(part 1 of 2)
# Autodesk Inventor assembly: ELEV_000_FULLASMBLY
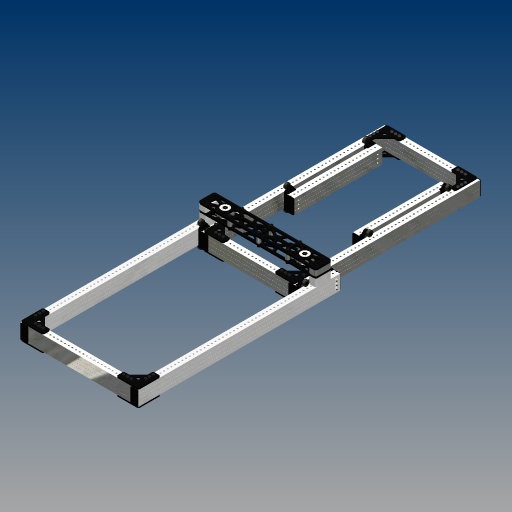
[picture p0: Inventor's stored thumbnail of the model, 512x512]
Saved by Autodesk Inventor 2024.3 (Build 283343000, 343)
## iProperties
Created: 2024-11-25
Part Number: ELEV_000_FULLASMBLY
Document SubType Name: Assembly
Designer: Kenji
Mass: 3407.89 g
Surface Area: 12378 cm^2
Volume: 1206.36 cm^3
Density: 2.82493 g/cm^3
Author: Kenji
## Documents named in this file (36)
- C:\Users\Kenji\Documents\GitHub\1622-2024-Casino-Clash-CAD-A-Thon\Elevator\ELEV_000_FULLASMBLY.iam
- C:\Users\Kenji\Documents\GitHub\1622-2024-Casino-Clash-CAD-A-Thon\Elevator\ELEV_001_BAR1(27.500 in).ipt
- C:\Users\Kenji\Documents\GitHub\1622-2024-Casino-Clash-CAD-A-Thon\Elevator\ELEV_002_BAR2(14.000 in).ipt
- C:\Users\Kenji\Documents\GitHub\1622-2024-Casino-Clash-CAD-A-Thon\Elevator\ELEV_003_BAR3(25.000 in).ipt
- C:\Users\Kenji\Documents\GitHub\1622-2024-Casino-Clash-CAD-A-Thon\COTS Library\Motion\BearingBlocks\ElevatorBlocks\WCP-0897_InlineBearingBlock.iam
- C:\Users\Kenji\Documents\GitHub\1622-2024-Casino-Clash-CAD-A-Thon\Elevator\ELEV_004_BAR4(12.000 in).ipt
- C:\Users\Kenji\Documents\GitHub\1622-2024-Casino-Clash-CAD-A-Thon\Elevator\ELEV_005_SUPBRK1.ipt
- C:\Users\Kenji\Documents\GitHub\1622-2024-Casino-Clash-CAD-A-Thon\COTS Library\Fasteners\Nuts\COTS_90633A411_Low-Strength Steel Thin Nylon-Insert Locknut_10-32.ipt
- C:\Users\Kenji\Documents\GitHub\1622-2024-Casino-Clash-CAD-A-Thon\Elevator\ELEV_006_SUPBRK1_THRD.ipt
- C:\Users\Kenji\Documents\GitHub\1622-2024-Casino-Clash-CAD-A-Thon\COTS Library\Fasteners\Bolts\Socket-Head\10-32\COTS_90044A121_Black-Oxide Alloy Steel Socket Head Screw_10-32_2.5in.ipt
- C:\Users\Kenji\Documents\GitHub\1622-2024-Casino-Clash-CAD-A-Thon\COTS Library\Fasteners\Bolts\Socket-Head\10-32\COTS_90044A202_Black-Oxide Alloy Steel Socket Head Screw_1-.375.ipt
- C:\Users\Kenji\Documents\GitHub\1622-2024-Casino-Clash-CAD-A-Thon\COTS Library\Fasteners\Bolts\Socket-Head\10-32\COTS_91251A342_Black-Oxide Alloy Steel Socket Head Screw_.5in.ipt
- C:\Users\Kenji\Documents\GitHub\1622-2024-Casino-Clash-CAD-A-Thon\Elevator\ELEV_007_SUPBRK2.ipt
- C:\Users\Kenji\Documents\GitHub\1622-2024-Casino-Clash-CAD-A-Thon\COTS Library\Fasteners\Bolts\Socket-Head\10-32\COTS_91251A359_Black-Oxide Alloy Steel Socket Head Screw_10-32_2_3-4in.ipt
- C:\Users\Kenji\Documents\GitHub\1622-2024-Casino-Clash-CAD-A-Thon\COTS Library\Fasteners\Nuts\COTS_90631A411_Low-Strength Steel Nylon-Insert Locknut_10-32.ipt
- C:\Users\Kenji\Documents\GitHub\1622-2024-Casino-Clash-CAD-A-Thon\Elevator\ELEV_008_SUPBRK3.ipt
- C:\Users\Kenji\Documents\GitHub\1622-2024-Casino-Clash-CAD-A-Thon\Elevator\ELEV_010_BOLTCOVER2.ipt
- C:\Users\Kenji\Documents\GitHub\1622-2024-Casino-Clash-CAD-A-Thon\Elevator\ELEV_011_EXTRUENDCAP.ipt
- C:\Users\Kenji\Documents\GitHub\1622-2024-Casino-Clash-CAD-A-Thon\Elevator\ELEV_012_SUPBRK2_THRD.ipt
- C:\Users\Kenji\Documents\GitHub\1622-2024-Casino-Clash-CAD-A-Thon\Elevator\ELEV_013_BAR5(12.000 in).ipt
- C:\Users\Kenji\Documents\GitHub\1622-2024-Casino-Clash-CAD-A-Thon\Elevator\ELEV_015_CRSHBLCK1.ipt
- C:\Users\Kenji\Documents\GitHub\1622-2024-Casino-Clash-CAD-A-Thon\Elevator\ELEV_019_SUPBAR3.ipt
- C:\Users\Kenji\Documents\GitHub\1622-2024-Casino-Clash-CAD-A-Thon\COTS Library\Motion\Bearings\COTS_WCP-0783_1.125ODHexBearing.ipt
- C:\Users\Kenji\Documents\GitHub\1622-2024-Casino-Clash-CAD-A-Thon\COTS Library\Motion\Sprockets\COTS_WCP-0974_#35_15t.ipt
- C:\Users\Kenji\Documents\GitHub\1622-2024-Casino-Clash-CAD-A-Thon\Elevator\ELEV_020_BILLET1(Shit).ipt
- C:\Users\Kenji\Documents\GitHub\1622-2024-Casino-Clash-CAD-A-Thon\Elevator\ELEV_021_SPACER2.ipt
- C:\Users\Kenji\Documents\GitHub\1622-2024-Casino-Clash-CAD-A-Thon\Elevator\ELEV_022_WASHER1(3DP).ipt
- C:\Users\Kenji\Documents\GitHub\1622-2024-Casino-Clash-CAD-A-Thon\COTS Library\Fasteners\Bolts\Socket-Head\0.25-20\COTS_91251A537_Black-Oxide Alloy Steel Socket Head Screw_.25-20_.5in.ipt
- C:\Users\Kenji\Documents\GitHub\1622-2024-Casino-Clash-CAD-A-Thon\Elevator\ELEV_023_BILLET2.ipt
- C:\Users\Kenji\Documents\GitHub\1622-2024-Casino-Clash-CAD-A-Thon\Elevator\ELEV_024_SPACER1.ipt
- C:\Users\Kenji\Documents\GitHub\1622-2024-Casino-Clash-CAD-A-Thon\Elevator\ELEV_000_FULLASMBLY\AIP\FEA\ew6g7bhkw.fins
- C:\Users\Kenji\Documents\GitHub\1622-2024-Casino-Clash-CAD-A-Thon\Elevator\ELEV_000_FULLASMBLY\AIP\FEA\ew6g7bhkw.fsat
- C:\Users\Kenji\Documents\GitHub\1622-2024-Casino-Clash-CAD-A-Thon\Elevator\ELEV_000_FULLASMBLY\AIP\FEA\ew6g7bhkw.ftes
- C:\Users\Kenji\Documents\GitHub\1622-2024-Casino-Clash-CAD-A-Thon\Elevator\ELEV_000_FULLASMBLY\AIP\FEA\ew6g7bhkw.fwiz
- C:\Users\Kenji\Documents\GitHub\1622-2024-Casino-Clash-CAD-A-Thon\Elevator\ELEV_000_FULLASMBLY\AIP\FEA\ew6g7biao.fmsh
- C:\Users\Kenji\Documents\GitHub\1622-2024-Casino-Clash-CAD-A-Thon\Elevator\ELEV_000_FULLASMBLY\AIP\FEA\ew6g7bibk.fres
## Components (210 placed, 29 different names)
1. ELEV_001_BAR1(27.500 in):1 — Flush:1, Flush:2, Mate:1, Mate:2, Flush:7, Tangent:2, Mate:10, Flush:11, Mate:11, Mate:78, Mate:133, Mate:136, Mate:137, Mate:201, Mate:202, Mate:203, Mate:284, Mate:285, Mate:286, Flush:35, Mate:341, Mate:359
2. ELEV_001_BAR1(27.500 in):2 — Flush:1, Flush:2, Mate:1, Flush:3, Flush:4, Mate:3, Angle:1, Mate:4, Flush:8, Angle:2, Mate:74, Mate:128, Mate:131, Mate:198, Mate:199, Mate:200, Mate:287, Mate:288, Mate:289, Mate:363
3. ELEV_002_BAR2(14.000 in):1 — Flush:3, Flush:4, Mate:2, Mate:127, Flush:24, Mate:132, Mate:134, Mate:135
4. ELEV_003_BAR3(25.000 in):1 — Flush:5, Flush:6, Flush:7, Mate:8, Flush:10, Mate:9, Mate:82, Mate:186, Mate:187, Mate:188, Mate:211, Mate:228, Tangent:3, Tangent:4, Angle:5, Angle:6, Mate:265, Mate:266, Mate:267
5. ELEV_003_BAR3(25.000 in):2 — Flush:5, Flush:6, Tangent:1, Angle:2, Mate:5, Angle:3, Mate:6, Flush:9, Mate:12, Flush:12, Flush:13, Mate:13, Flush:14, Mate:14, Mate:16, Mate:62, Mate:86, Mate:189, Mate:190, Mate:191, Mate:192, Mate:193, Mate:194, Mate:207, Mate:208, Tangent:5, Flush:33
6. WCP-0897_InlineBearingBlock:1 [sub-assembly] — Mate:5, Angle:3, Mate:6, Flush:9, Mate:83, Mate:84
7. WCP-0897_InlineBearingBlock:2 [sub-assembly] — Mate:3, Angle:1, Mate:4, Tangent:1, Flush:8, Mate:71, Mate:72
8. WCP-0897_InlineBearingBlock:3 [sub-assembly] — Mate:8, Flush:10, Mate:9, Tangent:2, Mate:79, Mate:80
9. WCP-0897_InlineBearingBlock:4 [sub-assembly] — Mate:10, Flush:11, Mate:11, Mate:75, Mate:76
10. ELEV_004_BAR4(12.000 in):1 — Mate:12, Flush:12, Flush:13, Mate:17, Mate:18, Mate:19, Angle:4, Mate:20, Mate:42, Mate:45, Mate:60, Flush:15, Mate:61
11. ELEV_004_BAR4(12.000 in):2 — Mate:13, Flush:14, Mate:14, Flush:26, Flush:27, Mate:214, Mate:227, Flush:28, Angle:7
12. ELEV_005_SUPBRK1:1 — Mate:16, Mate:17, Mate:18, Mate:67, Mate:68, Mate:69, Mate:70
13. ELEV_005_SUPBRK1:2 — Mate:19, Angle:4, Mate:20, Mate:63, Mate:64, Mate:65, Mate:66
14. ELEV_006_SUPBRK1_THRD:1 — Mate:42, Mate:61, Mate:62, Mate:247, Mate:248
15. ELEV_006_SUPBRK1_THRD:2 — Mate:45, Mate:60, Flush:15, Mate:241, Mate:242, Mate:243, Mate:244
16. ELEV_008_SUPBRK3:1 — Mate:127, Flush:24, Mate:128, Mate:129, Mate:130, Mate:138, Mate:139, Mate:144, Mate:145
17. ELEV_008_SUPBRK3:2 — Mate:129, Mate:130, Mate:131, Mate:148, Mate:149
18. ELEV_008_SUPBRK3:3 — Mate:132, Mate:133, Mate:134, Mate:151, Mate:153
19. ELEV_008_SUPBRK3:4 — Mate:135, Mate:136, Mate:137, Mate:140, Mate:141, Mate:142, Mate:143
20. ELEV_011_EXTRUENDCAP:1 — Mate:189, Mate:190, Mate:191
21. ELEV_011_EXTRUENDCAP:3 — Mate:186, Mate:187, Mate:188
22. ELEV_011_EXTRUENDCAP:5 — Mate:198, Mate:199, Mate:200
23. ELEV_011_EXTRUENDCAP:6 — Mate:201, Mate:202, Mate:203
24. ELEV_011_EXTRUENDCAP:7 — Mate:192, Mate:193, Mate:194
25. ELEV_007_SUPBRK2:1 — Flush:26, Mate:227, Mate:228, Mate:229, Mate:230, Mate:231, Mate:232, Mate:233
26. ELEV_007_SUPBRK2:2 — Flush:27, Mate:207, Mate:208, Mate:212, Mate:213, Mate:217, Mate:218, Mate:219, Mate:220
27. ELEV_012_SUPBRK2_THRD:1 — Mate:211, Mate:229, Flush:28, Mate:239, Mate:240
28. ELEV_012_SUPBRK2_THRD:2 — Mate:212, Mate:213, Mate:214, Mate:235, Mate:332
29. ELEV_013_BAR5(12.000 in):1 — Mate:257, Flush:29, Mate:258, Mate:259, Flush:30, Mate:260, Angle:5, Angle:6, Flush:34, Mate:277, Mate:283, Mate:333, Mate:334, Mate:335
30. ELEV_013_BAR5(12.000 in):2 — Mate:261, Flush:31, Mate:262, Mate:263, Flush:32, Mate:264, Angle:7, Flush:33, Flush:34, Mate:279, Mate:281, Mate:336, Mate:337, Mate:338
31. WCP-0897_InlineBearingBlock:5 [sub-assembly] — Mate:257, Flush:29, Mate:258, Tangent:3, Tangent:4, Mate:270, Mate:271
32. WCP-0897_InlineBearingBlock:6 [sub-assembly] — Mate:259, Flush:30, Mate:260, Mate:274, Mate:275
33. WCP-0897_InlineBearingBlock:7 [sub-assembly] — Mate:261, Flush:31, Mate:262, Tangent:5, Mate:272, Mate:273
34. WCP-0897_InlineBearingBlock:8 [sub-assembly] — Mate:263, Flush:32, Mate:264, Mate:268, Mate:269
35. ELEV_011_EXTRUENDCAP:8 — Mate:265, Mate:266, Mate:267
36. ELEV_015_CRSHBLCK1:1 — Mate:284, Mate:285, Mate:286
37. ELEV_015_CRSHBLCK1:2 — Mate:287, Mate:288, Mate:289
38. ELEV_011_EXTRUENDCAP:9 — Mate:333, Mate:334, Mate:335
39. ELEV_011_EXTRUENDCAP:10 — Mate:336, Mate:337, Mate:338
40. ELEV_019_SUPBAR3:1 — Flush:35, Mate:341, Mate:342, Mate:343, Mate:344, Mate:345, Mate:348, Mate:349, Mate:357, Mate:358, Mate:364, Mate:365, Mate:366, Mate:367, Mate:368, Mate:369, Mate:370, Mate:371, Mate:374, Mate:386, Mate:387, Mate:388, Mate:389, Mate:390, Mate:391, Mate:392, Mate:393, Mate:394, Mate:395, Mate:396, Mate:397, Mate:410, Mate:411, Mate:412, Mate:415
41. ELEV_019_SUPBAR3:2 — Mate:342, Mate:343, Mate:346, Mate:347, Mate:350, Mate:351, Mate:360, Mate:361, Mate:362, Mate:372, Mate:373, Mate:375, Mate:376, Mate:398, Mate:399, Mate:400, Mate:401, Mate:402, Mate:403, Mate:404, Mate:405, Mate:406, Mate:407, Mate:408, Mate:409, Mate:413, Mate:414
42. COTS_WCP-0783_1.125ODHexBearing:1 — Mate:347, Mate:350, Mate:352, Angle:11, Mate:383
43. COTS_WCP-0783_1.125ODHexBearing:2 — Mate:345, Mate:349, Angle:10, Mate:380, Mate:381, Mate:382, Mate:417, Angle:13, Flush:37
44. COTS_WCP-0783_1.125ODHexBearing:3 — Mate:346, Mate:351, Angle:9
45. COTS_WCP-0783_1.125ODHexBearing:4 — Mate:344, Mate:348, Mate:353, Angle:8, Mate:378, Mate:416, Angle:12, Flush:36
46. COTS_WCP-0974_#35_15t:1 — Mate:352, Angle:10, Angle:11, Mate:385
47. COTS_WCP-0974_#35_15t:2 — Mate:353, Angle:8, Angle:9, Mate:377, Mate:379, Mate:384
48. ELEV_020_BILLET1(Shit):1 — Mate:357, Mate:358, Mate:359, Mate:360
49. ELEV_020_BILLET1(Shit):2 — Mate:361, Mate:362, Mate:363
50. ELEV_021_SPACER2:1 — Mate:368, Mate:371
51. ELEV_021_SPACER2:2 — Mate:367, Mate:375
52. ELEV_021_SPACER2:3 — Mate:366, Mate:374, Mate:376
53. ELEV_021_SPACER2:4 — Mate:365, Mate:373
54. ELEV_021_SPACER2:5 — Mate:364, Mate:372
55. ELEV_021_SPACER2:6 — Mate:369, Mate:370
56. ELEV_022_WASHER1(3DP):1 — Mate:381, Mate:382, Mate:385
57. ELEV_022_WASHER1(3DP):2 — Mate:380, Mate:383
58. ELEV_022_WASHER1(3DP):3 — Mate:377, Mate:378
59. ELEV_022_WASHER1(3DP):4 — Mate:379, Mate:384
60. COTS_91251A537_Black-Oxide Alloy Steel Socket Head Screw_.25-20_.5in:1 — Mate:386, Mate:396
61. COTS_91251A537_Black-Oxide Alloy Steel Socket Head Screw_.25-20_.5in:2 — Mate:387, Mate:397
62. COTS_91251A537_Black-Oxide Alloy Steel Socket Head Screw_.25-20_.5in:3 — Mate:388, Mate:394
63. COTS_91251A537_Black-Oxide Alloy Steel Socket Head Screw_.25-20_.5in:4 — Mate:389, Mate:395
64. COTS_91251A537_Black-Oxide Alloy Steel Socket Head Screw_.25-20_.5in:5 — Mate:390, Mate:392
65. COTS_91251A537_Black-Oxide Alloy Steel Socket Head Screw_.25-20_.5in:6 — Mate:391, Mate:393
66. COTS_91251A537_Black-Oxide Alloy Steel Socket Head Screw_.25-20_.5in:7 — Mate:399, Mate:405
67. COTS_91251A537_Black-Oxide Alloy Steel Socket Head Screw_.25-20_.5in:8 — Mate:400, Mate:406
68. COTS_91251A537_Black-Oxide Alloy Steel Socket Head Screw_.25-20_.5in:9 — Mate:401, Mate:407
69. COTS_91251A537_Black-Oxide Alloy Steel Socket Head Screw_.25-20_.5in:10 — Mate:402, Mate:408
70. COTS_91251A537_Black-Oxide Alloy Steel Socket Head Screw_.25-20_.5in:11 — Mate:398, Mate:404
71. COTS_91251A537_Black-Oxide Alloy Steel Socket Head Screw_.25-20_.5in:12 — Mate:403, Mate:409
72. ELEV_023_BILLET2:1 — Mate:410, Mate:411, Mate:412
73. ELEV_023_BILLET2:2 — Mate:413, Mate:414, Mate:415
74. ELEV_024_SPACER1:1 — Mate:416, Angle:12, Flush:36
75. ELEV_024_SPACER1:2 — Mate:417, Angle:13, Flush:37
76. COTS_90044A121_Black-Oxide Alloy Steel Socket Head Screw_10-32_2.5in:1 — Mate:63, Mate:64
77. COTS_90044A121_Black-Oxide Alloy Steel Socket Head Screw_10-32_2.5in:5
78. COTS_90044A121_Black-Oxide Alloy Steel Socket Head Screw_10-32_2.5in:6
79. COTS_90044A121_Black-Oxide Alloy Steel Socket Head Screw_10-32_2.5in:4 — Mate:65, Mate:66
80. COTS_90044A121_Black-Oxide Alloy Steel Socket Head Screw_10-32_2.5in:7
81. COTS_90044A121_Black-Oxide Alloy Steel Socket Head Screw_10-32_2.5in:8
82. COTS_90044A121_Black-Oxide Alloy Steel Socket Head Screw_10-32_2.5in:2 — Mate:67, Mate:69, Mate:245
83. COTS_90044A121_Black-Oxide Alloy Steel Socket Head Screw_10-32_2.5in:11
84. COTS_90044A121_Black-Oxide Alloy Steel Socket Head Screw_10-32_2.5in:12
85. COTS_90044A202_Black-Oxide Alloy Steel Socket Head Screw_1-.375:1 — Mate:71, Mate:72, Mate:73
86. COTS_90633A411_Low-Strength Steel Thin Nylon-Insert Locknut_10-32:1 — Mate:73, Mate:74
87. COTS_90044A202_Black-Oxide Alloy Steel Socket Head Screw_1-.375:2
88. COTS_90633A411_Low-Strength Steel Thin Nylon-Insert Locknut_10-32:2
89. COTS_90044A202_Black-Oxide Alloy Steel Socket Head Screw_1-.375:3
90. COTS_90633A411_Low-Strength Steel Thin Nylon-Insert Locknut_10-32:3
91. COTS_90633A411_Low-Strength Steel Thin Nylon-Insert Locknut_10-32:4 — Mate:77, Mate:78
92. COTS_90044A202_Black-Oxide Alloy Steel Socket Head Screw_1-.375:4 — Mate:75, Mate:76, Mate:77
93. COTS_90633A411_Low-Strength Steel Thin Nylon-Insert Locknut_10-32:5
94. COTS_90044A202_Black-Oxide Alloy Steel Socket Head Screw_1-.375:5
95. COTS_90633A411_Low-Strength Steel Thin Nylon-Insert Locknut_10-32:6
96. COTS_90044A202_Black-Oxide Alloy Steel Socket Head Screw_1-.375:6
97. COTS_91251A342_Black-Oxide Alloy Steel Socket Head Screw_.5in:1 — Mate:79, Mate:80, Mate:81
98. COTS_90633A411_Low-Strength Steel Thin Nylon-Insert Locknut_10-32:7 — Mate:81, Mate:82
99. COTS_91251A342_Black-Oxide Alloy Steel Socket Head Screw_.5in:2
100. COTS_90633A411_Low-Strength Steel Thin Nylon-Insert Locknut_10-32:8
101. COTS_91251A342_Black-Oxide Alloy Steel Socket Head Screw_.5in:3
102. COTS_90633A411_Low-Strength Steel Thin Nylon-Insert Locknut_10-32:9
103. COTS_90633A411_Low-Strength Steel Thin Nylon-Insert Locknut_10-32:10 — Mate:85, Mate:86
104. COTS_91251A342_Black-Oxide Alloy Steel Socket Head Screw_.5in:4 — Mate:83, Mate:84, Mate:85
105. COTS_90633A411_Low-Strength Steel Thin Nylon-Insert Locknut_10-32:11
106. COTS_91251A342_Black-Oxide Alloy Steel Socket Head Screw_.5in:5
107. COTS_90633A411_Low-Strength Steel Thin Nylon-Insert Locknut_10-32:12
108. COTS_91251A342_Black-Oxide Alloy Steel Socket Head Screw_.5in:6
109. COTS_90631A411_Low-Strength Steel Nylon-Insert Locknut_10-32:14 — Mate:152, Mate:153, Mate:255
110. COTS_91251A359_Black-Oxide Alloy Steel Socket Head Screw_10-32_2_3-4in:14 — Mate:140, Mate:143, Mate:152, Mate:249
111. COTS_90631A411_Low-Strength Steel Nylon-Insert Locknut_10-32:17
112. COTS_91251A359_Black-Oxide Alloy Steel Socket Head Screw_10-32_2_3-4in:17
113. COTS_90631A411_Low-Strength Steel Nylon-Insert Locknut_10-32:18
114. COTS_91251A359_Black-Oxide Alloy Steel Socket Head Screw_10-32_2_3-4in:18
115. COTS_91251A359_Black-Oxide Alloy Steel Socket Head Screw_10-32_2_3-4in:13 — Mate:141, Mate:142, Mate:150, Mate:250
116. COTS_90631A411_Low-Strength Steel Nylon-Insert Locknut_10-32:15 — Mate:150, Mate:151, Mate:256
117. COTS_91251A359_Black-Oxide Alloy Steel Socket Head Screw_10-32_2_3-4in:19
118. COTS_90631A411_Low-Strength Steel Nylon-Insert Locknut_10-32:19
119. COTS_91251A359_Black-Oxide Alloy Steel Socket Head Screw_10-32_2_3-4in:20
120. COTS_90631A411_Low-Strength Steel Nylon-Insert Locknut_10-32:20
121. COTS_91251A359_Black-Oxide Alloy Steel Socket Head Screw_10-32_2_3-4in:15 — Mate:139, Mate:145, Mate:147
122. COTS_90631A411_Low-Strength Steel Nylon-Insert Locknut_10-32:13 — Mate:147, Mate:149
123. COTS_91251A359_Black-Oxide Alloy Steel Socket Head Screw_10-32_2_3-4in:21
124. COTS_90631A411_Low-Strength Steel Nylon-Insert Locknut_10-32:21
125. COTS_91251A359_Black-Oxide Alloy Steel Socket Head Screw_10-32_2_3-4in:22 — Mate:251
126. COTS_90631A411_Low-Strength Steel Nylon-Insert Locknut_10-32:22 — Mate:254
127. COTS_90631A411_Low-Strength Steel Nylon-Insert Locknut_10-32:16 — Mate:146, Mate:148, Mate:253
128. COTS_91251A359_Black-Oxide Alloy Steel Socket Head Screw_10-32_2_3-4in:16 — Mate:138, Mate:144, Mate:146, Mate:252
129. COTS_90631A411_Low-Strength Steel Nylon-Insert Locknut_10-32:23
130. COTS_91251A359_Black-Oxide Alloy Steel Socket Head Screw_10-32_2_3-4in:23
131. COTS_90631A411_Low-Strength Steel Nylon-Insert Locknut_10-32:24
132. COTS_91251A359_Black-Oxide Alloy Steel Socket Head Screw_10-32_2_3-4in:24
133. COTS_90044A121_Black-Oxide Alloy Steel Socket Head Screw_10-32_2.5in:15 — Mate:230, Mate:233, Mate:237
134. ELEV_010_BOLTCOVER2:28 — Mate:237, Mate:240
135. COTS_90044A121_Black-Oxide Alloy Steel Socket Head Screw_10-32_2.5in:17
136. ELEV_010_BOLTCOVER2:29
137. COTS_90044A121_Black-Oxide Alloy Steel Socket Head Screw_10-32_2.5in:18
138. ELEV_010_BOLTCOVER2:30
139. ELEV_010_BOLTCOVER2:26 — Mate:238, Mate:239
140. COTS_90044A121_Black-Oxide Alloy Steel Socket Head Screw_10-32_2.5in:14 — Mate:231, Mate:232, Mate:238
141. ELEV_010_BOLTCOVER2:31
142. COTS_90044A121_Black-Oxide Alloy Steel Socket Head Screw_10-32_2.5in:19
143. ELEV_010_BOLTCOVER2:32
144. COTS_90044A121_Black-Oxide Alloy Steel Socket Head Screw_10-32_2.5in:20
145. COTS_90044A121_Black-Oxide Alloy Steel Socket Head Screw_10-32_2.5in:13 — Mate:217, Mate:220, Mate:234
146. ELEV_010_BOLTCOVER2:25 — Mate:234, Mate:235
147. COTS_90044A121_Black-Oxide Alloy Steel Socket Head Screw_10-32_2.5in:21
148. ELEV_010_BOLTCOVER2:33
149. COTS_90044A121_Black-Oxide Alloy Steel Socket Head Screw_10-32_2.5in:22
150. ELEV_010_BOLTCOVER2:34
151. COTS_90044A121_Black-Oxide Alloy Steel Socket Head Screw_10-32_2.5in:16 — Mate:218, Mate:219, Mate:236, Mate:331
152. ELEV_010_BOLTCOVER2:27 — Mate:236
153. COTS_90044A121_Black-Oxide Alloy Steel Socket Head Screw_10-32_2.5in:23
154. ELEV_010_BOLTCOVER2:35
155. COTS_90044A121_Black-Oxide Alloy Steel Socket Head Screw_10-32_2.5in:24
156. ELEV_010_BOLTCOVER2:36
157. ELEV_010_BOLTCOVER2:38 — Mate:242, Mate:243
158. ELEV_010_BOLTCOVER2:41
159. ELEV_010_BOLTCOVER2:42
160. ELEV_010_BOLTCOVER2:37 — Mate:241, Mate:244
161. ELEV_010_BOLTCOVER2:43
162. ELEV_010_BOLTCOVER2:44
163. ELEV_010_BOLTCOVER2:40 — Mate:245, Mate:248
164. ELEV_010_BOLTCOVER2:45
165. ELEV_010_BOLTCOVER2:46
166. ELEV_010_BOLTCOVER2:39 — Mate:246, Mate:247
167. COTS_90044A121_Black-Oxide Alloy Steel Socket Head Screw_10-32_2.5in:3 — Mate:68, Mate:70, Mate:246
168. ELEV_010_BOLTCOVER2:47
169. COTS_90044A121_Black-Oxide Alloy Steel Socket Head Screw_10-32_2.5in:25
170. ELEV_010_BOLTCOVER2:48
171. COTS_90044A121_Black-Oxide Alloy Steel Socket Head Screw_10-32_2.5in:26
172. ELEV_010_BOLTCOVER2:50 — Mate:250, Mate:256
173. ELEV_010_BOLTCOVER2:53
174. ELEV_010_BOLTCOVER2:54
175. ELEV_010_BOLTCOVER2:49 — Mate:249, Mate:255
176. ELEV_010_BOLTCOVER2:55
177. ELEV_010_BOLTCOVER2:56
178. ELEV_010_BOLTCOVER2:51 — Mate:251, Mate:254
179. ELEV_010_BOLTCOVER2:57
180. ELEV_010_BOLTCOVER2:58
181. ELEV_010_BOLTCOVER2:52 — Mate:252, Mate:253
182. ELEV_010_BOLTCOVER2:59
183. ELEV_010_BOLTCOVER2:60
184. COTS_90633A411_Low-Strength Steel Thin Nylon-Insert Locknut_10-32:16 — Mate:282, Mate:283
185. COTS_91251A342_Black-Oxide Alloy Steel Socket Head Screw_.5in:7 — Mate:274, Mate:275, Mate:282
186. COTS_90633A411_Low-Strength Steel Thin Nylon-Insert Locknut_10-32:17
187. COTS_91251A342_Black-Oxide Alloy Steel Socket Head Screw_.5in:11
188. COTS_90633A411_Low-Strength Steel Thin Nylon-Insert Locknut_10-32:18
189. COTS_91251A342_Black-Oxide Alloy Steel Socket Head Screw_.5in:12
190. COTS_91251A342_Black-Oxide Alloy Steel Socket Head Screw_.5in:10 — Mate:270, Mate:271, Mate:276
191. COTS_90633A411_Low-Strength Steel Thin Nylon-Insert Locknut_10-32:13 — Mate:276, Mate:277
192. COTS_91251A342_Black-Oxide Alloy Steel Socket Head Screw_.5in:13
193. COTS_90633A411_Low-Strength Steel Thin Nylon-Insert Locknut_10-32:19
194. COTS_91251A342_Black-Oxide Alloy Steel Socket Head Screw_.5in:14
195. COTS_90633A411_Low-Strength Steel Thin Nylon-Insert Locknut_10-32:20
196. COTS_90633A411_Low-Strength Steel Thin Nylon-Insert Locknut_10-32:14 — Mate:278, Mate:279
197. COTS_91251A342_Black-Oxide Alloy Steel Socket Head Screw_.5in:9 — Mate:268, Mate:269, Mate:278
198. COTS_90633A411_Low-Strength Steel Thin Nylon-Insert Locknut_10-32:21
199. COTS_91251A342_Black-Oxide Alloy Steel Socket Head Screw_.5in:15
200. COTS_90633A411_Low-Strength Steel Thin Nylon-Insert Locknut_10-32:22
201. COTS_91251A342_Black-Oxide Alloy Steel Socket Head Screw_.5in:16
202. COTS_91251A342_Black-Oxide Alloy Steel Socket Head Screw_.5in:8 — Mate:272, Mate:273, Mate:280
203. COTS_90633A411_Low-Strength Steel Thin Nylon-Insert Locknut_10-32:15 — Mate:280, Mate:281
204. COTS_91251A342_Black-Oxide Alloy Steel Socket Head Screw_.5in:17
205. COTS_90633A411_Low-Strength Steel Thin Nylon-Insert Locknut_10-32:23
206. COTS_91251A342_Black-Oxide Alloy Steel Socket Head Screw_.5in:18
207. COTS_90633A411_Low-Strength Steel Thin Nylon-Insert Locknut_10-32:24
208. ELEV_010_BOLTCOVER2:61 — Mate:331, Mate:332
209. ELEV_010_BOLTCOVER2:62
210. ELEV_010_BOLTCOVER2:63
## Component patterns: (3 elements, first: COTS_90044A121_Black-Oxide Alloy Steel Socket Head Screw_10-32_2.5in:1), (3 elements, first: COTS_90044A121_Black-Oxide Alloy Steel Socket Head Screw_10-32_2.5in:4), (3 elements, first: COTS_90044A121_Black-Oxide Alloy Steel Socket Head Screw_10-32_2.5in:2), (3 elements, first: COTS_90044A202_Black-Oxide Alloy Steel Socket Head Screw_1-.375:1 + COTS_90633A411_Low-Strength Steel Thin Nylon-Insert Locknut_10-32:1), (3 elements, first: COTS_90633A411_Low-Strength Steel Thin Nylon-Insert Locknut_10-32:4 + COTS_90044A202_Black-Oxide Alloy Steel Socket Head Screw_1-.375:4), (3 elements, first: COTS_91251A342_Black-Oxide Alloy Steel Socket Head Screw_.5in:1 + COTS_90633A411_Low-Strength Steel Thin Nylon-Insert Locknut_10-32:7), (3 elements, first: COTS_90633A411_Low-Strength Steel Thin Nylon-Insert Locknut_10-32:10 + COTS_91251A342_Black-Oxide Alloy Steel Socket Head Screw_.5in:4), (3 elements, first: COTS_90631A411_Low-Strength Steel Nylon-Insert Locknut_10-32:14 + COTS_91251A359_Black-Oxide Alloy Steel Socket Head Screw_10-32_2_3-4in:14), (3 elements, first: COTS_91251A359_Black-Oxide Alloy Steel Socket Head Screw_10-32_2_3-4in:13 + COTS_90631A411_Low-Strength Steel Nylon-Insert Locknut_10-32:15), (3 elements, first: COTS_91251A359_Black-Oxide Alloy Steel Socket Head Screw_10-32_2_3-4in:15 + COTS_90631A411_Low-Strength Steel Nylon-Insert Locknut_10-32:13), (3 elements, first: COTS_90631A411_Low-Strength Steel Nylon-Insert Locknut_10-32:16 + COTS_91251A359_Black-Oxide Alloy Steel Socket Head Screw_10-32_2_3-4in:16), (3 elements, first: COTS_90044A121_Black-Oxide Alloy Steel Socket Head Screw_10-32_2.5in:15 + ELEV_010_BOLTCOVER2:28), (3 elements, first: ELEV_010_BOLTCOVER2:26 + COTS_90044A121_Black-Oxide Alloy Steel Socket Head Screw_10-32_2.5in:14), (3 elements, first: COTS_90044A121_Black-Oxide Alloy Steel Socket Head Screw_10-32_2.5in:13 + ELEV_010_BOLTCOVER2:25), (3 elements, first: COTS_90044A121_Black-Oxide Alloy Steel Socket Head Screw_10-32_2.5in:16 + ELEV_010_BOLTCOVER2:27), (3 elements, first: ELEV_010_BOLTCOVER2:38), (3 elements, first: ELEV_010_BOLTCOVER2:37), (3 elements, first: ELEV_010_BOLTCOVER2:40), (3 elements, first: ELEV_010_BOLTCOVER2:39 + COTS_90044A121_Black-Oxide Alloy Steel Socket Head Screw_10-32_2.5in:3), (3 elements, first: ELEV_010_BOLTCOVER2:50), (3 elements, first: ELEV_010_BOLTCOVER2:49), (3 elements, first: ELEV_010_BOLTCOVER2:51), (3 elements, first: ELEV_010_BOLTCOVER2:52), (3 elements, first: COTS_90633A411_Low-Strength Steel Thin Nylon-Insert Locknut_10-32:16 + COTS_91251A342_Black-Oxide Alloy Steel Socket Head Screw_.5in:7), (3 elements, first: COTS_91251A342_Black-Oxide Alloy Steel Socket Head Screw_.5in:10 + COTS_90633A411_Low-Strength Steel Thin Nylon-Insert Locknut_10-32:13), (3 elements, first: COTS_90633A411_Low-Strength Steel Thin Nylon-Insert Locknut_10-32:14 + COTS_91251A342_Black-Oxide Alloy Steel Socket Head Screw_.5in:9), (3 elements, first: COTS_91251A342_Black-Oxide Alloy Steel Socket Head Screw_.5in:8 + COTS_90633A411_Low-Strength Steel Thin Nylon-Insert Locknut_10-32:15), (3 elements, first: ELEV_010_BOLTCOVER2:61)
## Relationships (290: Mate 244, Flush 28, Angle 13, Tangent 5)
- Flush:1: ELEV_001_BAR1(27.500 in):1 ↔ ELEV_001_BAR1(27.500 in):2
- Flush:2: ELEV_001_BAR1(27.500 in):1 ↔ ELEV_001_BAR1(27.500 in):2
- Mate:1 (355.6 mm): ELEV_001_BAR1(27.500 in):1 ↔ ELEV_001_BAR1(27.500 in):2
- Flush:3: ELEV_001_BAR1(27.500 in):2 ↔ ELEV_002_BAR2(14.000 in):1
- Flush:4: ELEV_001_BAR1(27.500 in):2 ↔ ELEV_002_BAR2(14.000 in):1
- Mate:2: ELEV_001_BAR1(27.500 in):1 ↔ ELEV_002_BAR2(14.000 in):1
- Flush:5: ELEV_003_BAR3(25.000 in):1 ↔ ELEV_003_BAR3(25.000 in):2
- Flush:6: ELEV_003_BAR3(25.000 in):1 ↔ ELEV_003_BAR3(25.000 in):2
- Flush:7: ELEV_001_BAR1(27.500 in):1 ↔ ELEV_003_BAR3(25.000 in):1
- Mate:3: ELEV_001_BAR1(27.500 in):2 ↔ WCP-0897_InlineBearingBlock:2
- Angle:1 (0 deg): ELEV_001_BAR1(27.500 in):2 ↔ WCP-0897_InlineBearingBlock:2
- Mate:4: ELEV_001_BAR1(27.500 in):2 ↔ WCP-0897_InlineBearingBlock:2
- Tangent:1: ELEV_003_BAR3(25.000 in):2 ↔ WCP-0897_InlineBearingBlock:2
- Flush:8: ELEV_001_BAR1(27.500 in):2 ↔ WCP-0897_InlineBearingBlock:2
- Angle:2 (0 deg): ELEV_001_BAR1(27.500 in):2 ↔ ELEV_003_BAR3(25.000 in):2
- Mate:5: ELEV_003_BAR3(25.000 in):2 ↔ WCP-0897_InlineBearingBlock:1
- Angle:3 (0 deg): ELEV_003_BAR3(25.000 in):2 ↔ WCP-0897_InlineBearingBlock:1
- Mate:6: ELEV_003_BAR3(25.000 in):2 ↔ WCP-0897_InlineBearingBlock:1
- Flush:9: ELEV_003_BAR3(25.000 in):2 ↔ WCP-0897_InlineBearingBlock:1
- Mate:8: ELEV_003_BAR3(25.000 in):1 ↔ WCP-0897_InlineBearingBlock:3
- Flush:10: ELEV_003_BAR3(25.000 in):1 ↔ WCP-0897_InlineBearingBlock:3
- Mate:9: ELEV_003_BAR3(25.000 in):1 ↔ WCP-0897_InlineBearingBlock:3
- Tangent:2: ELEV_001_BAR1(27.500 in):1 ↔ WCP-0897_InlineBearingBlock:3
- Mate:10: ELEV_001_BAR1(27.500 in):1 ↔ WCP-0897_InlineBearingBlock:4
- Flush:11: ELEV_001_BAR1(27.500 in):1 ↔ WCP-0897_InlineBearingBlock:4
- Mate:11: ELEV_001_BAR1(27.500 in):1 ↔ WCP-0897_InlineBearingBlock:4
- Mate:12: ELEV_003_BAR3(25.000 in):2 ↔ ELEV_004_BAR4(12.000 in):1
- Flush:12: ELEV_003_BAR3(25.000 in):2 ↔ ELEV_004_BAR4(12.000 in):1
- Flush:13: ELEV_003_BAR3(25.000 in):2 ↔ ELEV_004_BAR4(12.000 in):1
- Mate:13: ELEV_003_BAR3(25.000 in):2 ↔ ELEV_004_BAR4(12.000 in):2
- Flush:14: ELEV_003_BAR3(25.000 in):2 ↔ ELEV_004_BAR4(12.000 in):2
- Mate:14: ELEV_003_BAR3(25.000 in):2 ↔ ELEV_004_BAR4(12.000 in):2
- Mate:16: ELEV_003_BAR3(25.000 in):2 ↔ ELEV_005_SUPBRK1:1
- Mate:17: ELEV_004_BAR4(12.000 in):1 ↔ ELEV_005_SUPBRK1:1
- Mate:18: ELEV_004_BAR4(12.000 in):1 ↔ ELEV_005_SUPBRK1:1
- Mate:19: ELEV_004_BAR4(12.000 in):1 ↔ ELEV_005_SUPBRK1:2
- Angle:4 (0 deg): ELEV_004_BAR4(12.000 in):1 ↔ ELEV_005_SUPBRK1:2
- Mate:20: ELEV_004_BAR4(12.000 in):1 ↔ ELEV_005_SUPBRK1:2
- Mate:42: ELEV_004_BAR4(12.000 in):1 ↔ ELEV_006_SUPBRK1_THRD:1
- Mate:45: ELEV_004_BAR4(12.000 in):1 ↔ ELEV_006_SUPBRK1_THRD:2
- Mate:60: ELEV_004_BAR4(12.000 in):1 ↔ ELEV_006_SUPBRK1_THRD:2
- Flush:15: ELEV_004_BAR4(12.000 in):1 ↔ ELEV_006_SUPBRK1_THRD:2
- Mate:61: ELEV_004_BAR4(12.000 in):1 ↔ ELEV_006_SUPBRK1_THRD:1
- Mate:62: ELEV_003_BAR3(25.000 in):2 ↔ ELEV_006_SUPBRK1_THRD:1
- Mate:63: ELEV_005_SUPBRK1:2 ↔ COTS_90044A121_Black-Oxide Alloy Steel Socket Head Screw_10-32_2.5in:1
- Mate:64: ELEV_005_SUPBRK1:2 ↔ COTS_90044A121_Black-Oxide Alloy Steel Socket Head Screw_10-32_2.5in:1
- Mate:65: ELEV_005_SUPBRK1:2 ↔ COTS_90044A121_Black-Oxide Alloy Steel Socket Head Screw_10-32_2.5in:4
- Mate:66: ELEV_005_SUPBRK1:2 ↔ COTS_90044A121_Black-Oxide Alloy Steel Socket Head Screw_10-32_2.5in:4
- Mate:67: ELEV_005_SUPBRK1:1 ↔ COTS_90044A121_Black-Oxide Alloy Steel Socket Head Screw_10-32_2.5in:2
- Mate:68: ELEV_005_SUPBRK1:1 ↔ COTS_90044A121_Black-Oxide Alloy Steel Socket Head Screw_10-32_2.5in:3
- Mate:69: ELEV_005_SUPBRK1:1 ↔ COTS_90044A121_Black-Oxide Alloy Steel Socket Head Screw_10-32_2.5in:2
- Mate:70: ELEV_005_SUPBRK1:1 ↔ COTS_90044A121_Black-Oxide Alloy Steel Socket Head Screw_10-32_2.5in:3
- Mate:71: WCP-0897_InlineBearingBlock:2 ↔ COTS_90044A202_Black-Oxide Alloy Steel Socket Head Screw_1-.375:1
- Mate:72: WCP-0897_InlineBearingBlock:2 ↔ COTS_90044A202_Black-Oxide Alloy Steel Socket Head Screw_1-.375:1
- Mate:73: COTS_90044A202_Black-Oxide Alloy Steel Socket Head Screw_1-.375:1 ↔ COTS_90633A411_Low-Strength Steel Thin Nylon-Insert Locknut_10-32:1
- Mate:74: ELEV_001_BAR1(27.500 in):2 ↔ COTS_90633A411_Low-Strength Steel Thin Nylon-Insert Locknut_10-32:1
- Mate:75: WCP-0897_InlineBearingBlock:4 ↔ COTS_90044A202_Black-Oxide Alloy Steel Socket Head Screw_1-.375:4
- Mate:76: WCP-0897_InlineBearingBlock:4 ↔ COTS_90044A202_Black-Oxide Alloy Steel Socket Head Screw_1-.375:4
- Mate:77: COTS_90633A411_Low-Strength Steel Thin Nylon-Insert Locknut_10-32:4 ↔ COTS_90044A202_Black-Oxide Alloy Steel Socket Head Screw_1-.375:4
- Mate:78: ELEV_001_BAR1(27.500 in):1 ↔ COTS_90633A411_Low-Strength Steel Thin Nylon-Insert Locknut_10-32:4
- Mate:79: WCP-0897_InlineBearingBlock:3 ↔ COTS_91251A342_Black-Oxide Alloy Steel Socket Head Screw_.5in:1
- Mate:80: WCP-0897_InlineBearingBlock:3 ↔ COTS_91251A342_Black-Oxide Alloy Steel Socket Head Screw_.5in:1
- Mate:81: COTS_91251A342_Black-Oxide Alloy Steel Socket Head Screw_.5in:1 ↔ COTS_90633A411_Low-Strength Steel Thin Nylon-Insert Locknut_10-32:7
- Mate:82: ELEV_003_BAR3(25.000 in):1 ↔ COTS_90633A411_Low-Strength Steel Thin Nylon-Insert Locknut_10-32:7
- Mate:83: WCP-0897_InlineBearingBlock:1 ↔ COTS_91251A342_Black-Oxide Alloy Steel Socket Head Screw_.5in:4
- Mate:84: WCP-0897_InlineBearingBlock:1 ↔ COTS_91251A342_Black-Oxide Alloy Steel Socket Head Screw_.5in:4
- Mate:85: COTS_90633A411_Low-Strength Steel Thin Nylon-Insert Locknut_10-32:10 ↔ COTS_91251A342_Black-Oxide Alloy Steel Socket Head Screw_.5in:4
- Mate:86: ELEV_003_BAR3(25.000 in):2 ↔ COTS_90633A411_Low-Strength Steel Thin Nylon-Insert Locknut_10-32:10
- Mate:127: ELEV_002_BAR2(14.000 in):1 ↔ ELEV_008_SUPBRK3:1
- Flush:24: ELEV_002_BAR2(14.000 in):1 ↔ ELEV_008_SUPBRK3:1
- Mate:128: ELEV_001_BAR1(27.500 in):2 ↔ ELEV_008_SUPBRK3:1
- Mate:129: ELEV_008_SUPBRK3:1 ↔ ELEV_008_SUPBRK3:2
- Mate:130: ELEV_008_SUPBRK3:1 ↔ ELEV_008_SUPBRK3:2
- Mate:131: ELEV_001_BAR1(27.500 in):2 ↔ ELEV_008_SUPBRK3:2
- Mate:132: ELEV_002_BAR2(14.000 in):1 ↔ ELEV_008_SUPBRK3:3
- Mate:133: ELEV_001_BAR1(27.500 in):1 ↔ ELEV_008_SUPBRK3:3
- Mate:134: ELEV_002_BAR2(14.000 in):1 ↔ ELEV_008_SUPBRK3:3
- Mate:135: ELEV_002_BAR2(14.000 in):1 ↔ ELEV_008_SUPBRK3:4
- Mate:136: ELEV_001_BAR1(27.500 in):1 ↔ ELEV_008_SUPBRK3:4
- Mate:137: ELEV_001_BAR1(27.500 in):1 ↔ ELEV_008_SUPBRK3:4
- Mate:138: ELEV_008_SUPBRK3:1 ↔ COTS_91251A359_Black-Oxide Alloy Steel Socket Head Screw_10-32_2_3-4in:16
- Mate:139: ELEV_008_SUPBRK3:1 ↔ COTS_91251A359_Black-Oxide Alloy Steel Socket Head Screw_10-32_2_3-4in:15
- Mate:140: ELEV_008_SUPBRK3:4 ↔ COTS_91251A359_Black-Oxide Alloy Steel Socket Head Screw_10-32_2_3-4in:14
- Mate:141: ELEV_008_SUPBRK3:4 ↔ COTS_91251A359_Black-Oxide Alloy Steel Socket Head Screw_10-32_2_3-4in:13
- Mate:142: ELEV_008_SUPBRK3:4 ↔ COTS_91251A359_Black-Oxide Alloy Steel Socket Head Screw_10-32_2_3-4in:13
- Mate:143: ELEV_008_SUPBRK3:4 ↔ COTS_91251A359_Black-Oxide Alloy Steel Socket Head Screw_10-32_2_3-4in:14
- Mate:144: ELEV_008_SUPBRK3:1 ↔ COTS_91251A359_Black-Oxide Alloy Steel Socket Head Screw_10-32_2_3-4in:16
- Mate:145: ELEV_008_SUPBRK3:1 ↔ COTS_91251A359_Black-Oxide Alloy Steel Socket Head Screw_10-32_2_3-4in:15
- Mate:146: COTS_90631A411_Low-Strength Steel Nylon-Insert Locknut_10-32:16 ↔ COTS_91251A359_Black-Oxide Alloy Steel Socket Head Screw_10-32_2_3-4in:16
- Mate:147: COTS_91251A359_Black-Oxide Alloy Steel Socket Head Screw_10-32_2_3-4in:15 ↔ COTS_90631A411_Low-Strength Steel Nylon-Insert Locknut_10-32:13
- Mate:148: ELEV_008_SUPBRK3:2 ↔ COTS_90631A411_Low-Strength Steel Nylon-Insert Locknut_10-32:16
- Mate:149: ELEV_008_SUPBRK3:2 ↔ COTS_90631A411_Low-Strength Steel Nylon-Insert Locknut_10-32:13
- Mate:150: COTS_91251A359_Black-Oxide Alloy Steel Socket Head Screw_10-32_2_3-4in:13 ↔ COTS_90631A411_Low-Strength Steel Nylon-Insert Locknut_10-32:15
- Mate:151: ELEV_008_SUPBRK3:3 ↔ COTS_90631A411_Low-Strength Steel Nylon-Insert Locknut_10-32:15
- Mate:152: COTS_90631A411_Low-Strength Steel Nylon-Insert Locknut_10-32:14 ↔ COTS_91251A359_Black-Oxide Alloy Steel Socket Head Screw_10-32_2_3-4in:14
- Mate:153: ELEV_008_SUPBRK3:3 ↔ COTS_90631A411_Low-Strength Steel Nylon-Insert Locknut_10-32:14
- Mate:186: ELEV_003_BAR3(25.000 in):1 ↔ ELEV_011_EXTRUENDCAP:3
- Mate:187: ELEV_003_BAR3(25.000 in):1 ↔ ELEV_011_EXTRUENDCAP:3
- Mate:188: ELEV_003_BAR3(25.000 in):1 ↔ ELEV_011_EXTRUENDCAP:3
- Mate:189: ELEV_003_BAR3(25.000 in):2 ↔ ELEV_011_EXTRUENDCAP:1
- Mate:190: ELEV_003_BAR3(25.000 in):2 ↔ ELEV_011_EXTRUENDCAP:1
- Mate:191: ELEV_003_BAR3(25.000 in):2 ↔ ELEV_011_EXTRUENDCAP:1
- Mate:192: ELEV_003_BAR3(25.000 in):2 ↔ ELEV_011_EXTRUENDCAP:7
- Mate:193: ELEV_003_BAR3(25.000 in):2 ↔ ELEV_011_EXTRUENDCAP:7
- Mate:194: ELEV_003_BAR3(25.000 in):2 ↔ ELEV_011_EXTRUENDCAP:7
- Mate:198: ELEV_001_BAR1(27.500 in):2 ↔ ELEV_011_EXTRUENDCAP:5
- Mate:199: ELEV_001_BAR1(27.500 in):2 ↔ ELEV_011_EXTRUENDCAP:5
- Mate:200: ELEV_001_BAR1(27.500 in):2 ↔ ELEV_011_EXTRUENDCAP:5
- Mate:201: ELEV_001_BAR1(27.500 in):1 ↔ ELEV_011_EXTRUENDCAP:6
- Mate:202: ELEV_001_BAR1(27.500 in):1 ↔ ELEV_011_EXTRUENDCAP:6
- Mate:203: ELEV_001_BAR1(27.500 in):1 ↔ ELEV_011_EXTRUENDCAP:6
- Flush:26: ELEV_004_BAR4(12.000 in):2 ↔ ELEV_007_SUPBRK2:1
- Flush:27: ELEV_004_BAR4(12.000 in):2 ↔ ELEV_007_SUPBRK2:2
- Mate:207: ELEV_003_BAR3(25.000 in):2 ↔ ELEV_007_SUPBRK2:2
- Mate:208: ELEV_003_BAR3(25.000 in):2 ↔ ELEV_007_SUPBRK2:2
- Mate:211: ELEV_003_BAR3(25.000 in):1 ↔ ELEV_012_SUPBRK2_THRD:1
- Mate:212: ELEV_007_SUPBRK2:2 ↔ ELEV_012_SUPBRK2_THRD:2
- Mate:213: ELEV_007_SUPBRK2:2 ↔ ELEV_012_SUPBRK2_THRD:2
- Mate:214: ELEV_004_BAR4(12.000 in):2 ↔ ELEV_012_SUPBRK2_THRD:2
- Mate:217: ELEV_007_SUPBRK2:2 ↔ COTS_90044A121_Black-Oxide Alloy Steel Socket Head Screw_10-32_2.5in:13
- Mate:218: ELEV_007_SUPBRK2:2 ↔ COTS_90044A121_Black-Oxide Alloy Steel Socket Head Screw_10-32_2.5in:16
- Mate:219: ELEV_007_SUPBRK2:2 ↔ COTS_90044A121_Black-Oxide Alloy Steel Socket Head Screw_10-32_2.5in:16
- Mate:220: ELEV_007_SUPBRK2:2 ↔ COTS_90044A121_Black-Oxide Alloy Steel Socket Head Screw_10-32_2.5in:13
- Mate:227: ELEV_004_BAR4(12.000 in):2 ↔ ELEV_007_SUPBRK2:1
- Mate:228: ELEV_003_BAR3(25.000 in):1 ↔ ELEV_007_SUPBRK2:1
- Mate:229: ELEV_007_SUPBRK2:1 ↔ ELEV_012_SUPBRK2_THRD:1
- Flush:28: ELEV_004_BAR4(12.000 in):2 ↔ ELEV_012_SUPBRK2_THRD:1
- Mate:230: ELEV_007_SUPBRK2:1 ↔ COTS_90044A121_Black-Oxide Alloy Steel Socket Head Screw_10-32_2.5in:15
- Mate:231: ELEV_007_SUPBRK2:1 ↔ COTS_90044A121_Black-Oxide Alloy Steel Socket Head Screw_10-32_2.5in:14
- Mate:232: ELEV_007_SUPBRK2:1 ↔ COTS_90044A121_Black-Oxide Alloy Steel Socket Head Screw_10-32_2.5in:14
- Mate:233: ELEV_007_SUPBRK2:1 ↔ COTS_90044A121_Black-Oxide Alloy Steel Socket Head Screw_10-32_2.5in:15
- Mate:234: COTS_90044A121_Black-Oxide Alloy Steel Socket Head Screw_10-32_2.5in:13 ↔ ELEV_010_BOLTCOVER2:25
- Mate:235: ELEV_012_SUPBRK2_THRD:2 ↔ ELEV_010_BOLTCOVER2:25
- Mate:236: COTS_90044A121_Black-Oxide Alloy Steel Socket Head Screw_10-32_2.5in:16 ↔ ELEV_010_BOLTCOVER2:27
- Mate:237: COTS_90044A121_Black-Oxide Alloy Steel Socket Head Screw_10-32_2.5in:15 ↔ ELEV_010_BOLTCOVER2:28
- Mate:238: ELEV_010_BOLTCOVER2:26 ↔ COTS_90044A121_Black-Oxide Alloy Steel Socket Head Screw_10-32_2.5in:14
- Mate:239: ELEV_012_SUPBRK2_THRD:1 ↔ ELEV_010_BOLTCOVER2:26
- Mate:240: ELEV_012_SUPBRK2_THRD:1 ↔ ELEV_010_BOLTCOVER2:28
- Mate:241: ELEV_006_SUPBRK1_THRD:2 ↔ ELEV_010_BOLTCOVER2:37
- Mate:242: ELEV_006_SUPBRK1_THRD:2 ↔ ELEV_010_BOLTCOVER2:38
- Mate:243: ELEV_006_SUPBRK1_THRD:2 ↔ ELEV_010_BOLTCOVER2:38
- Mate:244: ELEV_006_SUPBRK1_THRD:2 ↔ ELEV_010_BOLTCOVER2:37
- Mate:245: COTS_90044A121_Black-Oxide Alloy Steel Socket Head Screw_10-32_2.5in:2 ↔ ELEV_010_BOLTCOVER2:40
- Mate:246: ELEV_010_BOLTCOVER2:39 ↔ COTS_90044A121_Black-Oxide Alloy Steel Socket Head Screw_10-32_2.5in:3
- Mate:247: ELEV_006_SUPBRK1_THRD:1 ↔ ELEV_010_BOLTCOVER2:39
- Mate:248: ELEV_006_SUPBRK1_THRD:1 ↔ ELEV_010_BOLTCOVER2:40
- Mate:249: COTS_91251A359_Black-Oxide Alloy Steel Socket Head Screw_10-32_2_3-4in:14 ↔ ELEV_010_BOLTCOVER2:49
- Mate:250: COTS_91251A359_Black-Oxide Alloy Steel Socket Head Screw_10-32_2_3-4in:13 ↔ ELEV_010_BOLTCOVER2:50
- Mate:251: COTS_91251A359_Black-Oxide Alloy Steel Socket Head Screw_10-32_2_3-4in:22 ↔ ELEV_010_BOLTCOVER2:51
- Mate:252: COTS_91251A359_Black-Oxide Alloy Steel Socket Head Screw_10-32_2_3-4in:16 ↔ ELEV_010_BOLTCOVER2:52
- Mate:253: COTS_90631A411_Low-Strength Steel Nylon-Insert Locknut_10-32:16 ↔ ELEV_010_BOLTCOVER2:52
- Mate:254: COTS_90631A411_Low-Strength Steel Nylon-Insert Locknut_10-32:22 ↔ ELEV_010_BOLTCOVER2:51
- Mate:255: COTS_90631A411_Low-Strength Steel Nylon-Insert Locknut_10-32:14 ↔ ELEV_010_BOLTCOVER2:49
- Mate:256: COTS_90631A411_Low-Strength Steel Nylon-Insert Locknut_10-32:15 ↔ ELEV_010_BOLTCOVER2:50
- Mate:257: ELEV_013_BAR5(12.000 in):1 ↔ WCP-0897_InlineBearingBlock:5
- Flush:29: ELEV_013_BAR5(12.000 in):1 ↔ WCP-0897_InlineBearingBlock:5
- Mate:258: ELEV_013_BAR5(12.000 in):1 ↔ WCP-0897_InlineBearingBlock:5